# Autodesk Inventor assembly: Inverter Assembly
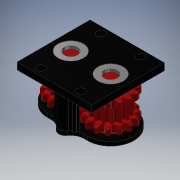
[picture p0: Inventor's stored thumbnail of the model, 180x180]
Saved by Autodesk Inventor 2019.4 (Build 234330000, 330)
## iProperties
Created: 2020-02-16
Part Number: Inverter Assembly
Document SubType Name: Assembly
Designer: admin
Author: admin
## Documents named in this file (5)
- C:\Users\admin\Desktop\FRC 2020 Engineering\GitHub\7738-2020\Robot V2\Storage System\3D printed Alternator\Inverter Assembly.iam
- C:\Users\admin\Desktop\FRC 2020 Engineering\GitHub\7738-2020\Robot V2\Storage System\3D printed Alternator\Alternator Axle.ipt
- C:\Users\admin\Desktop\FRC 2020 Engineering\GitHub\7738-2020\Robot V2\Storage System\3D printed Alternator\F6800.ipt
- C:\Users\admin\Desktop\FRC 2020 Engineering\GitHub\7738-2020\Robot V2\Storage System\3D printed Alternator\Inverter Housing Half 1.ipt
- C:\Users\admin\Desktop\FRC 2020 Engineering\GitHub\7738-2020\Robot V2\Storage System\3D printed Alternator\Inverter Housing Half 2.ipt
## Components (8 placed, 4 different names)
1. Alternator Axle:1 — Mate:1, Flush:1, Mate:2, Mate:5, Mate:6, Mate:8
2. Alternator Axle:2 — Mate:1, Flush:1, Mate:3, Mate:4, Mate:7, Mate:9
3. F6800:1 — Mate:4, Mate:7, Mate:11
4. F6800:2 — Mate:5, Mate:6, Mate:10, Mate:12
5. F6800:3 — Mate:3, Mate:9, Mate:13, Mate:14
6. F6800:4 — Mate:2, Mate:8, Mate:15
7. Inverter Housing Half 1:1 — Mate:10, Mate:11, Mate:12
8. Inverter Housing Half 2:1 — Mate:13, Mate:14, Mate:15
## Relationships (16: Mate 15, Flush 1)
- Mate:1 (30 mm): Alternator Axle:1 ↔ Alternator Axle:2
- Flush:1: Alternator Axle:1 ↔ Alternator Axle:2
- Mate:2: Alternator Axle:1 ↔ F6800:4
- Mate:3: Alternator Axle:2 ↔ F6800:3
- Mate:4: Alternator Axle:2 ↔ F6800:1
- Mate:5: Alternator Axle:1 ↔ F6800:2
- Mate:6 (0.2 mm): Alternator Axle:1 ↔ F6800:2
- Mate:7 (0.2 mm): Alternator Axle:2 ↔ F6800:1
- Mate:8 (0.2 mm): Alternator Axle:1 ↔ F6800:4
- Mate:9 (0.2 mm): Alternator Axle:2 ↔ F6800:3
- Mate:10: F6800:2 ↔ Inverter Housing Half 1:1
- Mate:11: F6800:1 ↔ Inverter Housing Half 1:1
- Mate:12: F6800:2 ↔ Inverter Housing Half 1:1
- Mate:13 (0.2 mm): F6800:3 ↔ Inverter Housing Half 2:1
- Mate:14: F6800:3 ↔ Inverter Housing Half 2:1
- Mate:15: F6800:4 ↔ Inverter Housing Half 2:1
